# Autodesk Inventor assembly: TLY装配整体
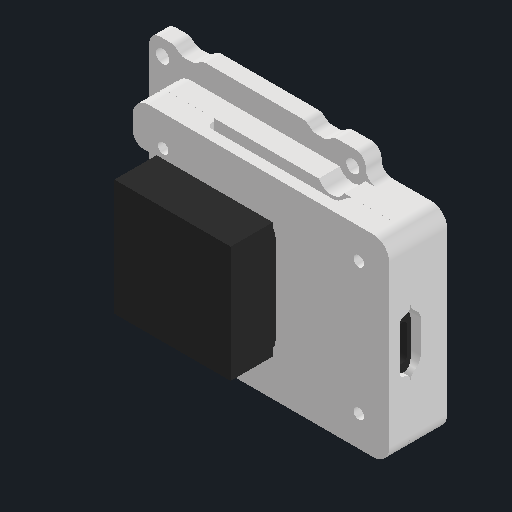
[picture p0: Inventor's stored thumbnail of the model, 512x512]
Saved by Autodesk Inventor 2025 (Build 290162000, 162)
## iProperties
Created: 2025-01-05
Part Number: TLY装配整体
Document SubType Name: Assembly
Designer: HZD
Author: HZD
## Documents named in this file (4)
- D:\2 B Mechanical design\GCG全向轮步兵\云台\TLY装配整体.iam
- D:\2 B Mechanical design\GCG全向轮步兵\云台\陀螺仪外壳.ipt
- D:\2 B Mechanical design\GCG全向轮步兵\云台\陀螺仪外壳2.ipt
- D:\2 B Mechanical design\GCG全向轮步兵\云台\陀螺仪.ipt
## Components (3 placed, 3 different names)
1. 陀螺仪外壳:1 — 配合:4, 配合:5, 配合:6
2. 陀螺仪外壳2:1 — 配合:1, 配合:2, 配合:3, 配合:4, 配合:5, 配合:6
3. 陀螺仪:1 — 配合:1, 配合:2, 配合:3
## Relationships (6: Mate 6)
- 配合:1 [Mate]: 陀螺仪外壳2:1 ↔ 陀螺仪:1
- 配合:2 [Mate]: 陀螺仪外壳2:1 ↔ 陀螺仪:1
- 配合:3 [Mate]: 陀螺仪外壳2:1 ↔ 陀螺仪:1
- 配合:4 [Mate]: 陀螺仪外壳:1 ↔ 陀螺仪外壳2:1
- 配合:5 [Mate]: 陀螺仪外壳:1 ↔ 陀螺仪外壳2:1
- 配合:6 [Mate]: 陀螺仪外壳:1 ↔ 陀螺仪外壳2:1
